# Autodesk Inventor assembly: one roller asmb_MIR
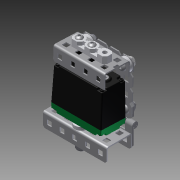
[picture p0: Inventor's stored thumbnail of the model, 180x180]
Saved by Autodesk Inventor 2014 SP1 (Build 180222100, 222)
## iProperties
Created: 2014-03-20
Part Number: one roller asmb_MIR
Document SubType Name: Assembly
Designer: Ryan
Author: Ryan
## Documents named in this file (17)
- C:\Users\Ryan\Desktop\sw\toss up 5th A bot\intake\one roller asmb_MIR.iam
- C:\Users\Ryan\Desktop\sw\lib\Aperture VEX CAD Library\Metal\C Channel\2 x 5.ipt
- C:\Users\Ryan\Desktop\sw\lib\Aperture VEX CAD Library\Metal\C Channel\2 x 4.ipt
- C:\Users\Ryan\Desktop\sw\lib\Aperture VEX CAD Library\Metal\Plate\4 x 4.ipt
- C:\Users\Ryan\Desktop\sw\lib\Aperture VEX CAD Library\Metal\vex hinge\hinge.iam
- C:\Users\Ryan\Desktop\sw\lib\Aperture VEX CAD Library\Hardware\8-32\8-32_.375.ipt
- C:\Users\Ryan\Desktop\sw\lib\Aperture VEX CAD Library\Hardware\8-32\8-32 nylock_MIR11.ipt
- C:\Users\Ryan\Desktop\sw\lib\Aperture VEX CAD Library\Hardware\8-32\8-32 nylock.ipt
- C:\Users\Ryan\Desktop\sw\lib\Aperture VEX CAD Library\Spacers\SPACER-0500-0125.ipt
- C:\Users\Ryan\Desktop\sw\lib\Aperture VEX CAD Library\Bearing Blocks\Bearing Block.ipt
- C:\Users\Ryan\Desktop\sw\lib\Aperture VEX CAD Library\Motors\2-Wire Motor 393-Without Wire.iam
- C:\Users\Ryan\Desktop\sw\lib\Aperture VEX CAD Library\Hardware\6-32\6-32_.500.ipt
- C:\Users\Ryan\Desktop\sw\lib\Aperture VEX CAD Library\Spacers\thin\SPACER-0320-0500.ipt
- C:\Users\Ryan\Desktop\sw\lib\Aperture VEX CAD Library\Hardware\8-32\8-32_.875.ipt
- C:\Users\Ryan\Desktop\sw\lib\Aperture VEX CAD Library\Spacers\thin\SPACER-0320-0125.ipt
- C:\Users\Ryan\Desktop\sw\lib\Aperture VEX CAD Library\Spacers\thin\SPACER-0320-0375.ipt
- C:\Users\Ryan\Desktop\sw\lib\Aperture VEX CAD Library\Hardware\8-32\8-23_.750.ipt
## Components (30 placed, 16 different names)
1. 2 x 5:1 — Mate:2, Flush:6, Flush:5, Mate:98, Mate:99, Mate:97, Mate:96, Mate:109, Mate:110, Mate:108, Mate:107, Mate:115, Mate:114, Mate:112, Mate:119, Flush:7
2. 2 x 4:1 — Flush:2, Flush:1, Mate:11, Mate:10, Mate:9, Mate:14, Mate:13, Mate:12, Mate:27, Mate:55, Mate:54, Mate:53, Mate:52, Mate:87
3. 4 x 4:1 — Flush:2, Flush:1, Flush:4, Flush:3, Mate:1, Mate:5, Mate:3, Mate:4, Mate:8, Mate:7, Mate:6, Mate:16, Mate:22, Mate:23, Mate:26, Flush:6
4. hinge:1 [sub-assembly] — Mate:2, Flush:6, Flush:5, Flush:4, Flush:3, Mate:1, Mate:21, Mate:20, Flush:6, Flush:7
5. 8-32_.375:1 — Mate:5, Mate:3, Mate:4, Mate:17
6. 8-32_.375:2 — Mate:8, Mate:7, Mate:6, Mate:18
7. 8-32_.375:3 — Mate:11, Mate:10, Mate:9, Mate:15, Mate:24
8. 8-32_.375:4 — Mate:14, Mate:13, Mate:12, Mate:19, Mate:25
9. 8-32 nylock_MIR11:1 — Mate:16, Mate:15
10. 8-32 nylock:1 — Mate:21, Mate:18
11. 8-32 nylock:2 — Mate:22, Mate:19
12. 8-32 nylock:3 — Mate:20, Mate:17
13. SPACER-0500-0125:1 — Mate:24, Mate:23
14. SPACER-0500-0125:2 — Mate:27, Mate:26, Mate:25
15. Bearing Block:1 — Mate:55, Mate:54, Mate:53, Mate:52, Mate:89, Mate:88, Mate:92, Mate:90, Mate:91
16. 2-Wire Motor 393-Without Wire:1 [sub-assembly] — Mate:89, Mate:88, Mate:87
17. 6-32_.500:1 — Mate:92, Mate:90, Flush:7
18. 6-32_.500:2 — Flush:7, Mate:91
19. SPACER-0500-0125:3 — Mate:98, Mate:94, Mate:93
20. SPACER-0320-0500:1 — Mate:99, Mate:95, Mate:100
21. 8-32_.875:1 — Mate:97, Mate:96, Mate:95, Mate:94, Mate:93, Mate:101
22. 8-32 nylock:4 — Mate:101, Mate:100
23. SPACER-0500-0125:4 — Mate:109, Mate:103, Mate:102
24. SPACER-0320-0500:2 — Mate:110, Mate:104, Mate:105
25. 8-32_.875:2 — Mate:108, Mate:107, Mate:104, Mate:103, Mate:102, Mate:106
26. 8-32 nylock:5 — Mate:106, Mate:105
27. SPACER-0320-0125:1 — Mate:113, Mate:111, Mate:117
28. SPACER-0320-0375:1 — Mate:115, Mate:114, Mate:113, Mate:112, Mate:111, Mate:116
29. 8-23_.750:1 — Mate:117, Mate:116, Mate:118
30. 8-32 nylock:6 — Mate:119, Mate:118
## Relationships (73: Mate 66, Flush 7)
- Flush:2: 2 x 4:1 ↔ 4 x 4:1
- Flush:1: 2 x 4:1 ↔ 4 x 4:1
- Mate:2: 2 x 5:1 ↔ hinge:1
- Flush:6: 2 x 5:1 ↔ hinge:1
- Flush:5 [Mate]: 2 x 5:1 ↔ hinge:1
- Flush:4: 4 x 4:1 ↔ hinge:1
- Flush:3 [Mate]: 4 x 4:1 ↔ hinge:1
- Mate:1: 4 x 4:1 ↔ hinge:1
- Mate:5: 4 x 4:1 ↔ 8-32_.375:1
- Mate:3 (2.3114 mm): 4 x 4:1 ↔ 8-32_.375:1
- Mate:4 (2.3114 mm): 4 x 4:1 ↔ 8-32_.375:1
- Mate:8: 4 x 4:1 ↔ 8-32_.375:2
- Mate:7 (2.3114 mm): 4 x 4:1 ↔ 8-32_.375:2
- Mate:6 (2.3114 mm): 4 x 4:1 ↔ 8-32_.375:2
- Mate:11 (2.3114 mm): 2 x 4:1 ↔ 8-32_.375:3
- Mate:10 (2.3114 mm): 2 x 4:1 ↔ 8-32_.375:3
- Mate:9: 2 x 4:1 ↔ 8-32_.375:3
- Mate:14: 2 x 4:1 ↔ 8-32_.375:4
- Mate:13 (2.3114 mm): 2 x 4:1 ↔ 8-32_.375:4
- Mate:12 (2.3114 mm): 2 x 4:1 ↔ 8-32_.375:4
- Mate:16: 4 x 4:1 ↔ 8-32 nylock_MIR11:1
- Mate:15: 8-32_.375:3 ↔ 8-32 nylock_MIR11:1
- Mate:21: hinge:1 ↔ 8-32 nylock:1
- Mate:18: 8-32_.375:2 ↔ 8-32 nylock:1
- Mate:22: 4 x 4:1 ↔ 8-32 nylock:2
- Mate:19: 8-32_.375:4 ↔ 8-32 nylock:2
- Mate:20: hinge:1 ↔ 8-32 nylock:3
- Mate:17: 8-32_.375:1 ↔ 8-32 nylock:3
- Mate:24: 8-32_.375:3 ↔ SPACER-0500-0125:1
- Mate:23: 4 x 4:1 ↔ SPACER-0500-0125:1
- Mate:27: 2 x 4:1 ↔ SPACER-0500-0125:2
- Mate:26: 4 x 4:1 ↔ SPACER-0500-0125:2
- Mate:25: 8-32_.375:4 ↔ SPACER-0500-0125:2
- Mate:55 (2.3114 mm): 2 x 4:1 ↔ Bearing Block:1
- Mate:54 (2.3114 mm): 2 x 4:1 ↔ Bearing Block:1
- Mate:53 (2.3114 mm): 2 x 4:1 ↔ Bearing Block:1
- Mate:52: 2 x 4:1 ↔ Bearing Block:1
- Mate:89: Bearing Block:1 ↔ 2-Wire Motor 393-Without Wire:1
- Mate:88: Bearing Block:1 ↔ 2-Wire Motor 393-Without Wire:1
- Mate:87: 2 x 4:1 ↔ 2-Wire Motor 393-Without Wire:1
- Mate:92: Bearing Block:1 ↔ 6-32_.500:1
- Mate:90: Bearing Block:1 ↔ 6-32_.500:1
- Flush:7: 6-32_.500:1 ↔ 6-32_.500:2
- Mate:91: Bearing Block:1 ↔ 6-32_.500:2
- Mate:98: 2 x 5:1 ↔ SPACER-0500-0125:3
- Mate:99: 2 x 5:1 ↔ SPACER-0320-0500:1
- Mate:97 (2.3114 mm): 2 x 5:1 ↔ 8-32_.875:1
- Mate:96 (2.3114 mm): 2 x 5:1 ↔ 8-32_.875:1
- Mate:95: SPACER-0320-0500:1 ↔ 8-32_.875:1
- Mate:94: SPACER-0500-0125:3 ↔ 8-32_.875:1
- Mate:93: SPACER-0500-0125:3 ↔ 8-32_.875:1
- Mate:101: 8-32_.875:1 ↔ 8-32 nylock:4
- Mate:100 (1.1684 mm): SPACER-0320-0500:1 ↔ 8-32 nylock:4
- Mate:109: 2 x 5:1 ↔ SPACER-0500-0125:4
- Mate:110: 2 x 5:1 ↔ SPACER-0320-0500:2
- Mate:108 (2.3114 mm): 2 x 5:1 ↔ 8-32_.875:2
- Mate:107 (2.3114 mm): 2 x 5:1 ↔ 8-32_.875:2
- Mate:104: SPACER-0320-0500:2 ↔ 8-32_.875:2
- Mate:103: SPACER-0500-0125:4 ↔ 8-32_.875:2
- Mate:102: SPACER-0500-0125:4 ↔ 8-32_.875:2
- Mate:106: 8-32_.875:2 ↔ 8-32 nylock:5
- Mate:105 (1.1684 mm): SPACER-0320-0500:2 ↔ 8-32 nylock:5
- Mate:115 (2.3114 mm): 2 x 5:1 ↔ SPACER-0320-0375:1
- Mate:114 (2.3114 mm): 2 x 5:1 ↔ SPACER-0320-0375:1
- Mate:113: SPACER-0320-0125:1 ↔ SPACER-0320-0375:1
- Mate:112: 2 x 5:1 ↔ SPACER-0320-0375:1
- Mate:111: SPACER-0320-0125:1 ↔ SPACER-0320-0375:1
- Mate:117: SPACER-0320-0125:1 ↔ 8-23_.750:1
- Mate:116: SPACER-0320-0375:1 ↔ 8-23_.750:1
- Mate:119: 2 x 5:1 ↔ 8-32 nylock:6
- Mate:118: 8-23_.750:1 ↔ 8-32 nylock:6
- Flush:6: 4 x 4:1 ↔ hinge:1
- Flush:7: 2 x 5:1 ↔ hinge:1
